# Autodesk Inventor assembly: HB_armMountU03
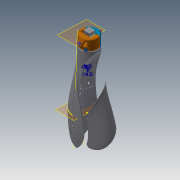
[picture p0: Inventor's stored thumbnail of the model, 180x180]
Saved by Autodesk Inventor 2015 SP1 (Build 190203100, 203)
## iProperties
Created: 2015-02-09
Part Number: HB_armMountU03
Document SubType Name: Assembly
Designer: Yamaura
Author: Yamaura
## Documents named in this file (30)
- C:\Users\Yamaura\Documents\GitHub\HACKberry\HACKberry-hardware\3D\Inventor\Parts\HB_armMountU03.iam
- C:\Users\Yamaura\Documents\GitHub\HACKberry\HACKberry-hardware\3D\Inventor\Parts\flatScrewM2L4PHI3.3T1.3.ipt
- C:\Users\Yamaura\Documents\GitHub\HACKberry\HACKberry-hardware\3D\Inventor\Parts\SBI-SUJ-1d4.ipt
- C:\Users\Yamaura\Documents\GitHub\HACKberry\HACKberry-hardware\3D\Inventor\Parts\CP 0.5-6-8.ipt
- C:\Users\Yamaura\Documents\GitHub\HACKberry\HACKberry-hardware\3D\Inventor\Parts\HBpronationLockPin02.ipt
- C:\Users\Yamaura\Documents\GitHub\HACKberry\HACKberry-hardware\3D\Inventor\Parts\HBlockPlateHolder02.ipt
- C:\Users\Yamaura\Documents\GitHub\HACKberry\HACKberry-hardware\3D\Inventor\Parts\HBwristMount01 v7.ipt
- C:\Users\Yamaura\Documents\GitHub\HACKberry\HACKberry-hardware\3D\Inventor\Parts\HBarmMountBaseCover02.ipt
- C:\Users\Yamaura\Documents\GitHub\HACKberry\HACKberry-hardware\3D\Inventor\Parts\HBabductionLever02.ipt
- C:\Users\Yamaura\Documents\GitHub\HACKberry\HACKberry-hardware\3D\Inventor\Parts\HBejectorLever02.ipt
- C:\Users\Yamaura\Documents\GitHub\HACKberry\HACKberry-hardware\3D\Inventor\Parts\HBarmMountBase02.ipt
- C:\Users\Yamaura\Documents\GitHub\HACKberry\HACKberry-hardware\3D\Inventor\Parts\HBarmMount02.ipt
- C:\Users\Yamaura\Documents\GitHub\HACKberry\HACKberry-hardware\3D\Inventor\Parts\HbBatteryDoor03.ipt
- C:\Users\Yamaura\Documents\GitHub\HACKberry\HACKberry-hardware\3D\Inventor\Parts\HbBatteryDoorKnob03.ipt
- C:\Users\Yamaura\Google ドライブ\exiii\3D\150405HackBerry\00_Latest\HbMainFrame03.ipt
- C:\Users\Yamaura\Documents\GitHub\HACKberry\HACKberry-hardware\3D\Inventor\Parts\HbBatteryHingeA03.ipt
- C:\Users\Yamaura\Documents\GitHub\HACKberry\HACKberry-hardware\3D\Inventor\Parts\HbBatteryHingeB03.ipt
- C:\Users\Yamaura\Documents\GitHub\HACKberry\HACKberry-hardware\3D\Inventor\Parts\HbBatteryHingeC03.ipt
- C:\Users\Yamaura\Documents\GitHub\HACKberry\HACKberry-hardware\3D\Inventor\Parts\HbBatteryCase01.ipt
- C:\Users\Yamaura\Documents\GitHub\HACKberry\HACKberry-hardware\3D\Inventor\Parts\HbBatteryLockKnob01.ipt
- C:\Users\Yamaura\Documents\GitHub\HACKberry\HACKberry-hardware\3D\Inventor\Parts\HbBatteryPcb01.ipt
- C:\Users\Yamaura\Documents\GitHub\HACKberry\HACKberry-hardware\3D\Inventor\Parts\DMW-BLF19.ipt
- C:\Users\Yamaura\Google ドライブ\exiii\3D\150405HackBerry\00_Latest\150404Morikawa.ipt
- C:\Users\Yamaura\Documents\GitHub\HACKberry\HACKberry-hardware\3D\Inventor\Parts\HbBatteryDoorLever03.ipt
- C:\Users\Yamaura\Documents\GitHub\HACKberry\HACKberry-hardware\3D\Inventor\Parts\HbMainFrameA01.ipt
- C:\Users\Yamaura\Documents\GitHub\HACKberry\HACKberry-hardware\3D\Inventor\Parts\HbMainFrameB01.ipt
- C:\Users\Yamaura\Documents\GitHub\HACKberry\HACKberry-hardware\3D\Inventor\Parts\HbUpperArmCover01.ipt
- C:\Users\Yamaura\Documents\GitHub\HACKberry\HACKberry-hardware\3D\Inventor\Parts\VN-3-1.ipt
- C:\Users\Yamaura\Documents\GitHub\HACKberry\HACKberry-hardware\3D\Inventor\Parts\ScrewM3L8Btite.ipt
- C:\Users\Yamaura\Google ドライブ\exiii\3D\150405HackBerry\00_Latest\flatScrewM2L4PHI3.3T1.3.ipt
## Components (42 placed, 28 different names)
1. flatScrewM2L4PHI3.3T1.3:1
2. flatScrewM2L4PHI3.3T1.3:2
3. SBI-SUJ-1d4:1
4. SBI-SUJ-1d4:2
5. CP 0.5-6-8:1 — メイト:56, メイト:57
6. CP 0.5-6-8:2
7. CP 0.5-6-8:3
8. CP 0.5-6-8:4
9. HBpronationLockPin02:1
10. HBlockPlateHolder02:1 — メイト:4, メイト:5, メイト:6, メイト:7
11. HBwristMount01 v7:1
12. HBarmMountBaseCover02:1 — メイト:65, メイト:66, メイト:67, メイト:68
13. HbMainFrame03:1 — メイト:3, メイト:4, メイト:5, メイト:6, 角度:1, メイト:10, メイト:22, メイト:23, メイト:24, メイト:25, メイト:26, メイト:27, メイト:28, メイト:31, メイト:43, メイト:48
14. HBabductionLever02:1 — メイト:41, 角度:2, メイト:42, メイト:56
15. HBejectorLever02:1 — メイト:57
16. HBarmMountBase02:1 — メイト:7, メイト:42
17. HBarmMount02:1
18. HbBatteryDoor03:1 — フラッシュ:5, メイト:44, メイト:45, メイト:46, メイト:47, メイト:48, メイト:49, メイト:50, メイト:51, 角度:3
19. HbBatteryHingeA03:1 — メイト:43, メイト:44, メイト:46
20. HbBatteryHingeB03:1 — メイト:31, メイト:40, メイト:45, メイト:47
21. HbBatteryHingeC03:1 — メイト:49, メイト:50, メイト:51
22. HbBatteryCase01:1 — メイト:22, メイト:23, メイト:29, メイト:30, メイト:34, メイト:35, メイト:36, フラッシュ:10, フラッシュ:11, フラッシュ:12, フラッシュ:13
23. HbBatteryLockKnob01:1 — メイト:24, メイト:25, メイト:30
24. HbBatteryPcb01:1 — メイト:26, メイト:27, メイト:28, メイト:29, メイト:61, メイト:62, メイト:63, メイト:64, メイト:69
25. DMW-BLF19:1 — メイト:34, メイト:35, メイト:36
26. 150404Morikawa:1
27. HbMainFrameA01:1 — フラッシュ:6, フラッシュ:7, フラッシュ:8, メイト:52, メイト:53, メイト:54
28. HbMainFrameB01:1 — メイト:52, メイト:53, メイト:54, メイト:70, メイト:71, メイト:72
29. HbUpperArmCover01:1 — メイト:55, フラッシュ:9
30. HbBatteryDoorKnob03:3 — メイト:58, メイト:59, メイト:60
31. VN-3-1:1 — メイト:61, メイト:64
32. VN-3-1:2 — メイト:62, メイト:63
33. ScrewM3L8Btite:1 — メイト:65, メイト:68
34. ScrewM3L8Btite:2 — メイト:66, メイト:67
35. flatScrewM2L4PHI3.3T1.3:3 — メイト:69, フラッシュ:10
36. flatScrewM2L4PHI3.3T1.3:4 — メイト:70, フラッシュ:12
37. flatScrewM2L4PHI3.3T1.3:5 — メイト:71, フラッシュ:13
38. flatScrewM2L4PHI3.3T1.3:6 — メイト:72, フラッシュ:11
39. HbBatteryDoorKnob03:1 — メイト:10, メイト:37, メイト:38, メイト:39
40. HbBatteryDoorKnob03:2
41. HbBatteryDoorLever03:1 — メイト:37, メイト:38, メイト:39, メイト:58, メイト:59, メイト:60
42. HbBatteryDoorLever03:2
## Component patterns: (2 elements, first: HbBatteryDoorKnob03:1), (2 elements, first: HbBatteryDoorLever03:1)
## Relationships (67: Mate 55, Flush 9, Angle 3)
- メイト:3 [Mate]: HbMainFrame03:1
- メイト:4 [Mate]: HBlockPlateHolder02:1 ↔ HbMainFrame03:1
- メイト:5 [Mate]: HBlockPlateHolder02:1 ↔ HbMainFrame03:1
- メイト:6 [Mate]: HBlockPlateHolder02:1 ↔ HbMainFrame03:1
- メイト:7 [Mate]: HBlockPlateHolder02:1 ↔ HBarmMountBase02:1
- 角度:1 [Angle] (90 deg): HbMainFrame03:1
- メイト:10 [Mate]: HbMainFrame03:1 ↔ HbBatteryDoorKnob03:1
- メイト:22 [Mate]: HbMainFrame03:1 ↔ HbBatteryCase01:1
- メイト:23 [Mate]: HbMainFrame03:1 ↔ HbBatteryCase01:1
- メイト:24 [Mate]: HbMainFrame03:1 ↔ HbBatteryLockKnob01:1
- メイト:25 [Mate] (0.1 mm): HbMainFrame03:1 ↔ HbBatteryLockKnob01:1
- メイト:26 [Mate]: HbMainFrame03:1 ↔ HbBatteryPcb01:1
- メイト:27 [Mate]: HbMainFrame03:1 ↔ HbBatteryPcb01:1
- メイト:28 [Mate] (0.1 mm): HbMainFrame03:1 ↔ HbBatteryPcb01:1
- メイト:29 [Mate]: HbBatteryCase01:1 ↔ HbBatteryPcb01:1
- メイト:30 [Mate]: HbBatteryCase01:1 ↔ HbBatteryLockKnob01:1
- メイト:31 [Mate]: HbMainFrame03:1 ↔ HbBatteryHingeB03:1
- メイト:34 [Mate]: HbBatteryCase01:1 ↔ DMW-BLF19:1
- メイト:35 [Mate]: HbBatteryCase01:1 ↔ DMW-BLF19:1
- メイト:36 [Mate] (0.1 mm): HbBatteryCase01:1 ↔ DMW-BLF19:1
- メイト:37 [Mate]: HbBatteryDoorKnob03:1 ↔ HbBatteryDoorLever03:1
- メイト:38 [Mate]: HbBatteryDoorKnob03:1 ↔ HbBatteryDoorLever03:1
- メイト:39 [Mate]: HbBatteryDoorKnob03:1 ↔ HbBatteryDoorLever03:1
- メイト:40 [Mate]: HbBatteryHingeB03:1
- フラッシュ:5 [Flush]: HbBatteryDoor03:1
- メイト:41 [Mate]: HBabductionLever02:1
- 角度:2 [Angle] (0 deg): HBabductionLever02:1
- メイト:42 [Mate]: HBabductionLever02:1 ↔ HBarmMountBase02:1
- メイト:43 [Mate]: HbMainFrame03:1 ↔ HbBatteryHingeA03:1
- メイト:44 [Mate]: HbBatteryDoor03:1 ↔ HbBatteryHingeA03:1
- メイト:45 [Mate]: HbBatteryDoor03:1 ↔ HbBatteryHingeB03:1
- メイト:46 [Mate]: HbBatteryDoor03:1 ↔ HbBatteryHingeA03:1
- メイト:47 [Mate]: HbBatteryDoor03:1 ↔ HbBatteryHingeB03:1
- メイト:48 [Mate] (0.2 mm): HbMainFrame03:1 ↔ HbBatteryDoor03:1
- メイト:49 [Mate]: HbBatteryDoor03:1 ↔ HbBatteryHingeC03:1
- メイト:50 [Mate]: HbBatteryDoor03:1 ↔ HbBatteryHingeC03:1
- メイト:51 [Mate]: HbBatteryDoor03:1 ↔ HbBatteryHingeC03:1
- 角度:3 [Angle] (0 deg): HbBatteryDoor03:1
- フラッシュ:6 [Flush] (-0.2 mm): HbMainFrameA01:1
- フラッシュ:7 [Flush]: HbMainFrameA01:1
- フラッシュ:8 [Flush]: HbMainFrameA01:1
- メイト:52 [Mate]: HbMainFrameA01:1 ↔ HbMainFrameB01:1
- メイト:53 [Mate]: HbMainFrameA01:1 ↔ HbMainFrameB01:1
- メイト:54 [Mate] (0.2 mm): HbMainFrameA01:1 ↔ HbMainFrameB01:1
- メイト:55 [Mate]: HbUpperArmCover01:1
- フラッシュ:9 [Flush]: HbUpperArmCover01:1
- メイト:56 [Mate]: CP 0.5-6-8:1 ↔ HBabductionLever02:1
- メイト:57 [Mate]: CP 0.5-6-8:1 ↔ HBejectorLever02:1
- メイト:58 [Mate]: HbBatteryDoorKnob03:3 ↔ HbBatteryDoorLever03:1
- メイト:59 [Mate]: HbBatteryDoorKnob03:3 ↔ HbBatteryDoorLever03:1
- メイト:60 [Mate]: HbBatteryDoorKnob03:3 ↔ HbBatteryDoorLever03:1
- メイト:61 [Mate]: HbBatteryPcb01:1 ↔ VN-3-1:1
- メイト:62 [Mate]: HbBatteryPcb01:1 ↔ VN-3-1:2
- メイト:63 [Mate]: HbBatteryPcb01:1 ↔ VN-3-1:2
- メイト:64 [Mate]: HbBatteryPcb01:1 ↔ VN-3-1:1
- メイト:65 [Mate]: HBarmMountBaseCover02:1 ↔ ScrewM3L8Btite:1
- メイト:66 [Mate]: HBarmMountBaseCover02:1 ↔ ScrewM3L8Btite:2
- メイト:67 [Mate]: HBarmMountBaseCover02:1 ↔ ScrewM3L8Btite:2
- メイト:68 [Mate]: HBarmMountBaseCover02:1 ↔ ScrewM3L8Btite:1
- メイト:69 [Mate]: HbBatteryPcb01:1 ↔ flatScrewM2L4PHI3.3T1.3:3
- フラッシュ:10 [Flush]: HbBatteryCase01:1 ↔ flatScrewM2L4PHI3.3T1.3:3
- メイト:70 [Mate]: HbMainFrameB01:1 ↔ flatScrewM2L4PHI3.3T1.3:4
- メイト:71 [Mate]: HbMainFrameB01:1 ↔ flatScrewM2L4PHI3.3T1.3:5
- メイト:72 [Mate]: HbMainFrameB01:1 ↔ flatScrewM2L4PHI3.3T1.3:6
- フラッシュ:11 [Flush]: HbBatteryCase01:1 ↔ flatScrewM2L4PHI3.3T1.3:6
- フラッシュ:12 [Flush]: HbBatteryCase01:1 ↔ flatScrewM2L4PHI3.3T1.3:4
- フラッシュ:13 [Flush]: HbBatteryCase01:1 ↔ flatScrewM2L4PHI3.3T1.3:5
